# Autodesk Inventor assembly: Bird_wing_assembly
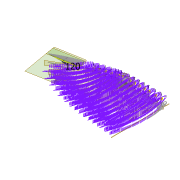
[picture p0: Inventor's stored thumbnail of the model, 180x180]
Saved by Autodesk Inventor 2022 (Build 260153000, 153)
## iProperties
Created: 2022-07-26
Part Number: Bird_wing_assembly
Document SubType Name: Assembly
Designer: dell
Mass: 478.578 g
Surface Area: 5047.89 cm^2
Volume: 478.578 cm^3
Density: 1 g/cm^3
Author: dell
## Documents named in this file (32)
- D:\xxxx\Uni\Part IV\MECHENG_700\Part_IV_project_CAD\Bird_skeleton_prototypes\Wing_drone_V1\Bird_wing_V2\Bird_wing_assembly.iam
- D:\xxxx\Uni\Part IV\MECHENG_700\Part_IV_project_CAD\Bird_skeleton_prototypes\Wing_drone_V1\Bird_wing_V2\Primary_hinge.ipt
- D:\xxxx\Uni\Part IV\MECHENG_700\Part_IV_project_CAD\Bird_skeleton_prototypes\Wing_drone_V1\Bird_wing_V2\Wing_arm_1.ipt
- D:\xxxx\Uni\Part IV\MECHENG_700\Part_IV_project_CAD\Bird_skeleton_prototypes\Wing_drone_V1\Bird_wing_V2\New_hinge_assembly.iam
- D:\xxxx\Uni\Part IV\MECHENG_700\Part_IV_project_CAD\Bird_skeleton_prototypes\Wing_drone_V1\Bird_wing_V2\Wing_arm_2.ipt
- D:\xxxx\Uni\Part IV\MECHENG_700\Part_IV_project_CAD\Bird_skeleton_prototypes\Wing_drone_V1\Bird_wing_V2\New_large_hinge_assembly.iam
- D:\xxxx\Uni\Part IV\MECHENG_700\Part_IV_project_CAD\Bird_skeleton_prototypes\Wing_drone_V1\Bird_wing_V2\Wing_arm_3.ipt
- D:\xxxx\Uni\Part IV\MECHENG_700\Part_IV_project_CAD\Bird_skeleton_prototypes\Wing_drone_V1\Bird_wing_V2\Arm_clip.ipt
- D:\xxxx\Uni\Part IV\MECHENG_700\Part_IV_project_CAD\Bird_skeleton_prototypes\Wing_drone_V1\Bird_wing_V2\Feather_clip.ipt
- D:\xxxx\Uni\Part IV\MECHENG_700\Part_IV_project_CAD\Bird_skeleton_prototypes\Wing_drone_V1\Bird_wing_V2\Feather_1\NACA_4412_300mm_feather_1_PLA.ipt
- D:\xxxx\Uni\Part IV\MECHENG_700\Part_IV_project_CAD\Bird_skeleton_prototypes\Wing_drone_V1\Bird_wing_V2\Feather_2\NACA_4412_300mm_feather_2_PLA.ipt
- D:\xxxx\Uni\Part IV\MECHENG_700\Part_IV_project_CAD\Bird_skeleton_prototypes\Wing_drone_V1\Bird_wing_V2\Feather_3\NACA_4412_340mm_feather_3_PLA.ipt
- D:\xxxx\Uni\Part IV\MECHENG_700\Part_IV_project_CAD\Bird_skeleton_prototypes\Wing_drone_V1\Bird_wing_V2\Feather_4\NACA_4412_340mm_feather_4_PLA.ipt
- D:\xxxx\Uni\Part IV\MECHENG_700\Part_IV_project_CAD\Bird_skeleton_prototypes\Wing_drone_V1\Bird_wing_V2\Feather_5\NACA_4412_340mm_feather_5_PLA.ipt
- D:\xxxx\Uni\Part IV\MECHENG_700\Part_IV_project_CAD\Bird_skeleton_prototypes\Wing_drone_V1\Bird_wing_V2\Feather_6\NACA_4412_340mm_feather_6_PLA.ipt
- D:\xxxx\Uni\Part IV\MECHENG_700\Part_IV_project_CAD\Bird_skeleton_prototypes\Wing_drone_V1\Bird_wing_V2\Feather_7\NACA_4412_340mm_feather_7_PLA.ipt
- D:\xxxx\Uni\Part IV\MECHENG_700\Part_IV_project_CAD\Bird_skeleton_prototypes\Wing_drone_V1\Bird_wing_V2\Feather_8\NACA_4412_340mm_feather_8_PLA.ipt
- D:\xxxx\Uni\Part IV\MECHENG_700\Part_IV_project_CAD\Bird_skeleton_prototypes\Wing_drone_V1\Bird_wing_V2\Feather_9\NACA_4412_340mm_feather_9_PLA.ipt
- D:\xxxx\Uni\Part IV\MECHENG_700\Part_IV_project_CAD\Bird_skeleton_prototypes\Wing_drone_V1\Bird_wing_V2\Feather_11\NACA_4412_340mm_feather_11_PLA.ipt
- D:\xxxx\Uni\Part IV\MECHENG_700\Part_IV_project_CAD\Bird_skeleton_prototypes\Wing_drone_V1\Bird_wing_V2\Feather_12\NACA_4412_340mm_feather_12_PLA.ipt
- D:\xxxx\Uni\Part IV\MECHENG_700\Part_IV_project_CAD\Bird_skeleton_prototypes\Wing_drone_V1\Bird_wing_V2\Feather_14\NACA_4412_340mm_feather_14_PLA.ipt
- D:\xxxx\Uni\Part IV\MECHENG_700\Part_IV_project_CAD\Bird_skeleton_prototypes\Wing_drone_V1\Bird_wing_V2\Feather_15\NACA_4412_340mm_feather_15_PLA.ipt
- D:\xxxx\Uni\Part IV\MECHENG_700\Part_IV_project_CAD\Bird_skeleton_prototypes\Wing_drone_V1\Bird_wing_V2\Feather_16\NACA_4412_340mm_feather_16_PLA.ipt
- D:\xxxx\Uni\Part IV\MECHENG_700\Part_IV_project_CAD\Bird_skeleton_prototypes\Wing_drone_V1\Bird_wing_V2\Feather_17\NACA_4412_340mm_feather_17_PLA.ipt
- D:\xxxx\Uni\Part IV\MECHENG_700\Part_IV_project_CAD\Bird_skeleton_prototypes\Wing_drone_V1\Bird_wing_V2\Wing_cover\Radius_joint_cover.ipt
- D:\xxxx\Uni\Part IV\MECHENG_700\Part_IV_project_CAD\Bird_skeleton_prototypes\Wing_drone_V1\Bird_wing_V2\Wing_cover\M4_nut.ipt
- D:\xxxx\Uni\Part IV\MECHENG_700\Part_IV_project_CAD\Bird_skeleton_prototypes\Wing_drone_V1\Bird_wing_V2\Wing_cover\Torsion_spring.ipt
- D:\xxxx\Uni\Part IV\MECHENG_700\Part_IV_project_CAD\Bird_skeleton_prototypes\Wing_drone_V1\Bird_wing_V2\Wing_cover\Manus_joint_cover.ipt
- D:\xxxx\Uni\Part IV\MECHENG_700\Part_IV_project_CAD\Bird_skeleton_prototypes\Wing_drone_V1\Bird_wing_V2\Wing_cover\Manus_joint_cover_2.ipt
- D:\xxxx\Uni\Part IV\MECHENG_700\Part_IV_project_CAD\Bird_skeleton_prototypes\Wing_drone_V1\Bird_wing_V2\Wing_cover\NACA_4412_500mm_cover.ipt
- D:\xxxx\Uni\Part IV\MECHENG_700\Part_IV_project_CAD\Bird_skeleton_prototypes\Wing_drone_V1\Bird_wing_V2\Primary_pulley_V2.ipt
- D:\xxxx\Uni\Part IV\MECHENG_700\Part_IV_project_CAD\Bird_skeleton_prototypes\Wing_drone_V1\Bird_wing_V2\Feather_0\Feather_0_assembly.iam
## Components (64 placed, 31 different names)
1. Primary_hinge:1 — Mate:1, Mate:2, Flush:1, Mate:3, Mate:4, Mate:5, Mate:158, Mate:160, Flush:31, Mate:179, Mate:180
2. Wing_arm_1:1 — Mate:3, Mate:4, Mate:5, Flush:10, Mate:67, Mate:68, Mate:108, Flush:27, Mate:109, Angle:19, Flush:29, Angle:20, Flush:30
3. Wing_arm_2:1 — Mate:14, Mate:16, Mate:15, Mate:69, Flush:11, Mate:70, Mate:87, Flush:13, Mate:89, Flush:15, Mate:90, Flush:16, Mate:106, Flush:21, Mate:107, Flush:22, Angle:12, Angle:14, Angle:15, Angle:17, Angle:18, Flush:33, Mate:168, Angle:26, Angle:28
4. New_hinge_assembly:3 [sub-assembly] — Mate:14, Mate:16, Mate:15, Mate:17, Mate:18, Angle:1, Flush:12, Flush:18, Flush:19, Flush:24, Flush:25, Angle:23
5. New_large_hinge_assembly:2 [sub-assembly] — Mate:17, Mate:18, Angle:1, Mate:19, Mate:20, Mate:21, Mate:39, Mate:40, Mate:46, Mate:51, Mate:52, Mate:58, Mate:62, Mate:66, Angle:21, Mate:164, Mate:165
6. Wing_arm_3:1 — Mate:19, Mate:20, Mate:21, Mate:25, Angle:2, Angle:3, Mate:38, Flush:3, Mate:43, Flush:4, Mate:47, Flush:5, Mate:50, Flush:6, Mate:55, Flush:7, Mate:61, Flush:8, Mate:65, Flush:9, Angle:5, Angle:6, Angle:7, Angle:8, Angle:9, Angle:10, Angle:11, Flush:32, Mate:181, Mate:182, Angle:27, Angle:28, Mate:185, Mate:186, Mate:187
7. Arm_clip:1 — Mate:25, Angle:2, Mate:27, Mate:28, Mate:39
8. Feather_clip:1 — Mate:27, Mate:28, Mate:35, Mate:36, Mate:37
9. NACA_4412_300mm_feather_1_PLA:1 — Mate:35, Mate:36, Mate:37, Angle:3
10. NACA_4412_340mm_feather_8_PLA:1 — Mate:125, Mate:126, Mate:127, Angle:11
11. Arm_clip:2 — Mate:38, Flush:3, Mate:40, Mate:41, Mate:42
12. Feather_clip:2 — Mate:41, Mate:42, Mate:73, Mate:74, Mate:75
13. Arm_clip:3 — Mate:43, Flush:4, Mate:44, Mate:45, Mate:46
14. Feather_clip:3 — Mate:44, Mate:45, Mate:110, Mate:111, Mate:112
15. Arm_clip:4 — Mate:47, Flush:5, Mate:48, Mate:49, Mate:51
16. Feather_clip:4 — Mate:48, Mate:49, Mate:113, Mate:114, Mate:115
17. Arm_clip:5 — Mate:50, Flush:6, Mate:52, Mate:53, Mate:54
18. Feather_clip:5 — Mate:53, Mate:54, Mate:116, Mate:117, Mate:118
19. Arm_clip:6 — Mate:55, Flush:7, Mate:56, Mate:57, Mate:58
20. Feather_clip:6 — Mate:56, Mate:57, Mate:119, Mate:120, Mate:121
21. Arm_clip:7 — Mate:61, Flush:8, Mate:62
22. Feather_clip:7 — Mate:122, Mate:123, Mate:124
23. Arm_clip:8 — Mate:65, Flush:9, Mate:66
24. Feather_clip:8 — Mate:125, Mate:126, Mate:127
25. New_hinge_assembly:4 [sub-assembly] — Flush:10, Mate:67, Mate:68, Mate:71, Mate:72, Angle:4, Mate:183, Mate:184
26. New_hinge_assembly:5 [sub-assembly] — Mate:69, Flush:11, Mate:70, Mate:71, Mate:72, Angle:4
27. NACA_4412_300mm_feather_2_PLA:1 — Mate:73, Mate:74, Mate:75, Angle:5
28. Arm_clip:9 — Mate:87, Flush:12, Flush:13
29. Feather_clip:9 — Mate:128, Mate:129, Mate:130
30. Arm_clip:11 — Mate:89, Flush:15, Flush:18
31. Feather_clip:11 — Mate:134, Mate:135, Mate:136
32. Arm_clip:12 — Mate:90, Flush:16, Flush:19
33. Feather_clip:12 — Mate:137, Mate:138, Mate:139
34. Arm_clip:14 — Mate:106, Flush:21, Flush:24
35. Feather_clip:14 — Mate:143, Mate:144, Mate:145
36. Arm_clip:15 — Mate:107, Flush:22, Flush:25
37. Feather_clip:15 — Mate:146, Mate:147, Mate:148
38. Arm_clip:16 — Mate:109, Flush:29, Mate:184
39. Feather_clip:16 — Mate:152, Mate:153, Mate:154
40. Arm_clip:17 — Mate:108, Flush:27, Mate:183
41. NACA_4412_340mm_feather_12_PLA:1 — Mate:137, Mate:138, Mate:139, Angle:15
42. Feather_clip:17 — Mate:149, Mate:150, Mate:151
43. NACA_4412_340mm_feather_3_PLA:1 — Mate:110, Mate:111, Mate:112, Angle:6
44. NACA_4412_340mm_feather_4_PLA:1 — Mate:113, Mate:114, Mate:115, Angle:7
45. NACA_4412_340mm_feather_5_PLA:1 — Mate:116, Mate:117, Mate:118, Angle:8
46. NACA_4412_340mm_feather_6_PLA:2 — Mate:119, Mate:120, Mate:121, Angle:9
47. NACA_4412_340mm_feather_7_PLA:1 — Mate:122, Mate:123, Mate:124, Angle:10
48. NACA_4412_340mm_feather_9_PLA:1 — Mate:128, Mate:129, Mate:130, Angle:12
49. NACA_4412_340mm_feather_11_PLA:1 — Mate:134, Mate:135, Mate:136, Angle:14
50. NACA_4412_340mm_feather_14_PLA:1 — Mate:143, Mate:144, Mate:145, Angle:17
51. NACA_4412_340mm_feather_15_PLA:1 — Mate:146, Mate:147, Mate:148, Angle:18
52. NACA_4412_340mm_feather_16_PLA:1 — Mate:149, Mate:150, Mate:151, Angle:19
53. NACA_4412_340mm_feather_17_PLA:1 — Mate:152, Mate:153, Mate:154, Angle:20
54. Radius_joint_cover:1 — Flush:30, Mate:160, Mate:161, Mate:178
55. M4_nut:1 — Mate:158
56. Torsion_spring:1 — Mate:161, Flush:31, Mate:178
57. Manus_joint_cover:1 — Angle:21, Flush:32, Mate:163, Mate:164
58. Manus_joint_cover_2:5 — Mate:165, Flush:33, Angle:23
59. NACA_4412_500mm_cover:1 — Mate:168, Angle:26
60. Primary_pulley_V2:1 — Mate:179, Mate:180
61. Feather_0_assembly:1 [sub-assembly] — Mate:181, Mate:182, Angle:27
62. NACA_4412_500mm_cover:2 — Mate:185
63. NACA_4412_500mm_cover:3 — Mate:187
64. NACA_4412_500mm_cover:4 — Mate:186
## Relationships (183: Mate 134, Flush 26, Angle 23)
- Mate:1: Primary_hinge:1
- Mate:2: Primary_hinge:1
- Flush:1: Primary_hinge:1
- Mate:3: Primary_hinge:1 ↔ Wing_arm_1:1
- Mate:4: Primary_hinge:1 ↔ Wing_arm_1:1
- Mate:5: Primary_hinge:1 ↔ Wing_arm_1:1
- Mate:14: Wing_arm_2:1 ↔ New_hinge_assembly:3
- Mate:16: Wing_arm_2:1 ↔ New_hinge_assembly:3
- Mate:15: Wing_arm_2:1 ↔ New_hinge_assembly:3
- Mate:17: New_hinge_assembly:3 ↔ New_large_hinge_assembly:2
- Mate:18 (0.1 mm): New_hinge_assembly:3 ↔ New_large_hinge_assembly:2
- Angle:1 (10 deg): New_hinge_assembly:3 ↔ New_large_hinge_assembly:2
- Mate:19: New_large_hinge_assembly:2 ↔ Wing_arm_3:1
- Mate:20: New_large_hinge_assembly:2 ↔ Wing_arm_3:1
- Mate:21: New_large_hinge_assembly:2 ↔ Wing_arm_3:1
- Mate:25: Wing_arm_3:1 ↔ Arm_clip:1
- Angle:2 (90 deg): Wing_arm_3:1 ↔ Arm_clip:1
- Mate:27: Arm_clip:1 ↔ Feather_clip:1
- Mate:28: Arm_clip:1 ↔ Feather_clip:1
- Mate:35: Feather_clip:1 ↔ NACA_4412_300mm_feather_1_PLA:1
- Mate:36: Feather_clip:1 ↔ NACA_4412_300mm_feather_1_PLA:1
- Mate:37 (0.1 mm): Feather_clip:1 ↔ NACA_4412_300mm_feather_1_PLA:1
- Angle:3 (160 deg): Wing_arm_3:1 ↔ NACA_4412_300mm_feather_1_PLA:1
- Mate:38: Wing_arm_3:1 ↔ Arm_clip:2
- Flush:3: Wing_arm_3:1 ↔ Arm_clip:2
- Mate:39 (310 mm): New_large_hinge_assembly:2 ↔ Arm_clip:1
- Mate:40 (260 mm): New_large_hinge_assembly:2 ↔ Arm_clip:2
- Mate:41: Arm_clip:2 ↔ Feather_clip:2
- Mate:42: Arm_clip:2 ↔ Feather_clip:2
- Mate:43: Wing_arm_3:1 ↔ Arm_clip:3
- Flush:4: Wing_arm_3:1 ↔ Arm_clip:3
- Mate:44: Arm_clip:3 ↔ Feather_clip:3
- Mate:45: Arm_clip:3 ↔ Feather_clip:3
- Mate:46 (210 mm): New_large_hinge_assembly:2 ↔ Arm_clip:3
- Mate:47: Wing_arm_3:1 ↔ Arm_clip:4
- Flush:5: Wing_arm_3:1 ↔ Arm_clip:4
- Mate:48: Arm_clip:4 ↔ Feather_clip:4
- Mate:49: Arm_clip:4 ↔ Feather_clip:4
- Mate:50: Wing_arm_3:1 ↔ Arm_clip:5
- Flush:6: Wing_arm_3:1 ↔ Arm_clip:5
- Mate:51 (160 mm): New_large_hinge_assembly:2 ↔ Arm_clip:4
- Mate:52 (110 mm): New_large_hinge_assembly:2 ↔ Arm_clip:5
- Mate:53: Arm_clip:5 ↔ Feather_clip:5
- Mate:54: Arm_clip:5 ↔ Feather_clip:5
- Mate:55: Wing_arm_3:1 ↔ Arm_clip:6
- Flush:7: Wing_arm_3:1 ↔ Arm_clip:6
- Mate:56: Arm_clip:6 ↔ Feather_clip:6
- Mate:57: Arm_clip:6 ↔ Feather_clip:6
- Mate:58 (70 mm): New_large_hinge_assembly:2 ↔ Arm_clip:6
- [Mate]: Arm_clip:7 ↔ Feather_clip:7
- [Mate]: Arm_clip:7 ↔ Feather_clip:7
- Mate:61: Wing_arm_3:1 ↔ Arm_clip:7
- Flush:8: Wing_arm_3:1 ↔ Arm_clip:7
- Mate:62 (40 mm): New_large_hinge_assembly:2 ↔ Arm_clip:7
- [Mate]: Arm_clip:8 ↔ Feather_clip:8
- [Mate]: Arm_clip:8 ↔ Feather_clip:8
- Mate:65: Wing_arm_3:1 ↔ Arm_clip:8
- Flush:9: Wing_arm_3:1 ↔ Arm_clip:8
- Mate:66 (10 mm): New_large_hinge_assembly:2 ↔ Arm_clip:8
- Flush:10: Wing_arm_1:1 ↔ New_hinge_assembly:4
- Mate:67: Wing_arm_1:1 ↔ New_hinge_assembly:4
- Mate:68: Wing_arm_1:1 ↔ New_hinge_assembly:4
- Mate:69: Wing_arm_2:1 ↔ New_hinge_assembly:5
- Flush:11: Wing_arm_2:1 ↔ New_hinge_assembly:5
- Mate:70: Wing_arm_2:1 ↔ New_hinge_assembly:5
- Mate:71: New_hinge_assembly:4 ↔ New_hinge_assembly:5
- Mate:72 (0.1 mm): New_hinge_assembly:4 ↔ New_hinge_assembly:5
- Angle:4 (0 deg): New_hinge_assembly:4 ↔ New_hinge_assembly:5
- Mate:73: Feather_clip:2 ↔ NACA_4412_300mm_feather_2_PLA:1
- Mate:74: Feather_clip:2 ↔ NACA_4412_300mm_feather_2_PLA:1
- Mate:75 (0.1 mm): Feather_clip:2 ↔ NACA_4412_300mm_feather_2_PLA:1
- Angle:5 (140 deg): Wing_arm_3:1 ↔ NACA_4412_300mm_feather_2_PLA:1
- [Mate]: Arm_clip:9 ↔ Feather_clip:9
- [Mate]: Arm_clip:9 ↔ Feather_clip:9
- [Mate]: Arm_clip:11 ↔ Feather_clip:11
- [Mate]: Arm_clip:11 ↔ Feather_clip:11
- [Mate]: Arm_clip:12 ↔ Feather_clip:12
- [Mate]: Arm_clip:12 ↔ Feather_clip:12
- Mate:87: Wing_arm_2:1 ↔ Arm_clip:9
- Flush:12 (-10 mm): New_hinge_assembly:3 ↔ Arm_clip:9
- Flush:13: Wing_arm_2:1 ↔ Arm_clip:9
- Mate:89: Wing_arm_2:1 ↔ Arm_clip:11
- Flush:15: Wing_arm_2:1 ↔ Arm_clip:11
- Mate:90: Wing_arm_2:1 ↔ Arm_clip:12
- Flush:16: Wing_arm_2:1 ↔ Arm_clip:12
- Flush:18 (-58 mm): New_hinge_assembly:3 ↔ Arm_clip:11
- Flush:19 (-106 mm): New_hinge_assembly:3 ↔ Arm_clip:12
- [Mate]: Arm_clip:14 ↔ Feather_clip:14
- [Mate]: Arm_clip:14 ↔ Feather_clip:14
- [Mate]: Arm_clip:15 ↔ Feather_clip:15
- [Mate]: Arm_clip:15 ↔ Feather_clip:15
- [Mate]: Arm_clip:16 ↔ Feather_clip:16
- [Mate]: Arm_clip:16 ↔ Feather_clip:16
- [Mate]: Arm_clip:17 ↔ Feather_clip:17
- [Mate]: Arm_clip:17 ↔ Feather_clip:17
- Mate:106: Wing_arm_2:1 ↔ Arm_clip:14
- Flush:21: Wing_arm_2:1 ↔ Arm_clip:14
- Mate:107: Wing_arm_2:1 ↔ Arm_clip:15
- Flush:22: Wing_arm_2:1 ↔ Arm_clip:15
- Flush:24 (-154 mm): New_hinge_assembly:3 ↔ Arm_clip:14
- Flush:25 (-202 mm): New_hinge_assembly:3 ↔ Arm_clip:15
- Mate:108: Wing_arm_1:1 ↔ Arm_clip:17
- Flush:27: Wing_arm_1:1 ↔ Arm_clip:17
- Mate:109: Wing_arm_1:1 ↔ Arm_clip:16
- Mate:110: Feather_clip:3 ↔ NACA_4412_340mm_feather_3_PLA:1
- Mate:111: Feather_clip:3 ↔ NACA_4412_340mm_feather_3_PLA:1
- Mate:112 (0.1 mm): Feather_clip:3 ↔ NACA_4412_340mm_feather_3_PLA:1
- Angle:6 (130 deg): Wing_arm_3:1 ↔ NACA_4412_340mm_feather_3_PLA:1
- Mate:113: Feather_clip:4 ↔ NACA_4412_340mm_feather_4_PLA:1
- Mate:114: Feather_clip:4 ↔ NACA_4412_340mm_feather_4_PLA:1
- Mate:115 (0.1 mm): Feather_clip:4 ↔ NACA_4412_340mm_feather_4_PLA:1
- Angle:7 (238 deg): Wing_arm_3:1 ↔ NACA_4412_340mm_feather_4_PLA:1
- Mate:116: Feather_clip:5 ↔ NACA_4412_340mm_feather_5_PLA:1
- Mate:117: Feather_clip:5 ↔ NACA_4412_340mm_feather_5_PLA:1
- Mate:118 (0.1 mm): Feather_clip:5 ↔ NACA_4412_340mm_feather_5_PLA:1
- Mate:119: Feather_clip:6 ↔ NACA_4412_340mm_feather_6_PLA:2
- Mate:120: Feather_clip:6 ↔ NACA_4412_340mm_feather_6_PLA:2
- Mate:121 (0.1 mm): Feather_clip:6 ↔ NACA_4412_340mm_feather_6_PLA:2
- Mate:122: Feather_clip:7 ↔ NACA_4412_340mm_feather_7_PLA:1
- Mate:123: Feather_clip:7 ↔ NACA_4412_340mm_feather_7_PLA:1
- Mate:124 (0.1 mm): Feather_clip:7 ↔ NACA_4412_340mm_feather_7_PLA:1
- Angle:8 (242 deg): Wing_arm_3:1 ↔ NACA_4412_340mm_feather_5_PLA:1
- Angle:9 (247 deg): Wing_arm_3:1 ↔ NACA_4412_340mm_feather_6_PLA:2
- Angle:10 (255 deg): Wing_arm_3:1 ↔ NACA_4412_340mm_feather_7_PLA:1
- Mate:125: NACA_4412_340mm_feather_8_PLA:1 ↔ Feather_clip:8
- Mate:126: NACA_4412_340mm_feather_8_PLA:1 ↔ Feather_clip:8
- Mate:127 (0.1 mm): NACA_4412_340mm_feather_8_PLA:1 ↔ Feather_clip:8
- Angle:11 (100 deg): Wing_arm_3:1 ↔ NACA_4412_340mm_feather_8_PLA:1
- Mate:128: Feather_clip:9 ↔ NACA_4412_340mm_feather_9_PLA:1
- Mate:129: Feather_clip:9 ↔ NACA_4412_340mm_feather_9_PLA:1
- Mate:130 (0.1 mm): Feather_clip:9 ↔ NACA_4412_340mm_feather_9_PLA:1
- Angle:12 (95 deg): Wing_arm_2:1 ↔ NACA_4412_340mm_feather_9_PLA:1
- Mate:134: Feather_clip:11 ↔ NACA_4412_340mm_feather_11_PLA:1
- Mate:135: Feather_clip:11 ↔ NACA_4412_340mm_feather_11_PLA:1
- Mate:136 (0.1 mm): Feather_clip:11 ↔ NACA_4412_340mm_feather_11_PLA:1
- Angle:14 (268 deg): Wing_arm_2:1 ↔ NACA_4412_340mm_feather_11_PLA:1
- Mate:137: Feather_clip:12 ↔ NACA_4412_340mm_feather_12_PLA:1
- Mate:138: Feather_clip:12 ↔ NACA_4412_340mm_feather_12_PLA:1
- Mate:139 (0.1 mm): Feather_clip:12 ↔ NACA_4412_340mm_feather_12_PLA:1
- Angle:15 (269 deg): Wing_arm_2:1 ↔ NACA_4412_340mm_feather_12_PLA:1
- Mate:143: Feather_clip:14 ↔ NACA_4412_340mm_feather_14_PLA:1
- Mate:144: Feather_clip:14 ↔ NACA_4412_340mm_feather_14_PLA:1
- Mate:145 (0.1 mm): Feather_clip:14 ↔ NACA_4412_340mm_feather_14_PLA:1
- Angle:17 (269 deg): Wing_arm_2:1 ↔ NACA_4412_340mm_feather_14_PLA:1
- Mate:146: Feather_clip:15 ↔ NACA_4412_340mm_feather_15_PLA:1
- Mate:147: Feather_clip:15 ↔ NACA_4412_340mm_feather_15_PLA:1
- Mate:148 (0.1 mm): Feather_clip:15 ↔ NACA_4412_340mm_feather_15_PLA:1
- Angle:18 (90 deg): Wing_arm_2:1 ↔ NACA_4412_340mm_feather_15_PLA:1
- Mate:149: Feather_clip:17 ↔ NACA_4412_340mm_feather_16_PLA:1
- Mate:150: Feather_clip:17 ↔ NACA_4412_340mm_feather_16_PLA:1
- Mate:151 (0.1 mm): Feather_clip:17 ↔ NACA_4412_340mm_feather_16_PLA:1
- Angle:19 (270 deg): Wing_arm_1:1 ↔ NACA_4412_340mm_feather_16_PLA:1
- Mate:152: Feather_clip:16 ↔ NACA_4412_340mm_feather_17_PLA:1
- Mate:153: Feather_clip:16 ↔ NACA_4412_340mm_feather_17_PLA:1
- Mate:154 (0.1 mm): Feather_clip:16 ↔ NACA_4412_340mm_feather_17_PLA:1
- Flush:29: Wing_arm_1:1 ↔ Arm_clip:16
- Angle:20 (90 deg): Wing_arm_1:1 ↔ NACA_4412_340mm_feather_17_PLA:1
- Mate:158: Primary_hinge:1 ↔ M4_nut:1
- Flush:30: Wing_arm_1:1 ↔ Radius_joint_cover:1
- Mate:160: Primary_hinge:1 ↔ Radius_joint_cover:1
- Mate:161: Radius_joint_cover:1 ↔ Torsion_spring:1
- Flush:31: Primary_hinge:1 ↔ Torsion_spring:1
- Angle:21 (10 deg): New_large_hinge_assembly:2 ↔ Manus_joint_cover:1
- Flush:32: Wing_arm_3:1 ↔ Manus_joint_cover:1
- Mate:163: Manus_joint_cover:1
- Mate:164: New_large_hinge_assembly:2 ↔ Manus_joint_cover:1
- Mate:165: New_large_hinge_assembly:2 ↔ Manus_joint_cover_2:5
- Flush:33: Wing_arm_2:1 ↔ Manus_joint_cover_2:5
- Angle:23 (-60 deg): New_hinge_assembly:3 ↔ Manus_joint_cover_2:5
- Mate:168: Wing_arm_2:1 ↔ NACA_4412_500mm_cover:1
- Angle:26 (0 deg): Wing_arm_2:1 ↔ NACA_4412_500mm_cover:1
- Mate:178: Radius_joint_cover:1 ↔ Torsion_spring:1
- Mate:179: Primary_hinge:1 ↔ Primary_pulley_V2:1
- Mate:180: Primary_hinge:1 ↔ Primary_pulley_V2:1
- Mate:181: Wing_arm_3:1 ↔ Feather_0_assembly:1
- Mate:182: Wing_arm_3:1 ↔ Feather_0_assembly:1
- Angle:27 (0 deg): Wing_arm_3:1 ↔ Feather_0_assembly:1
- Mate:183 (12 mm): New_hinge_assembly:4 ↔ Arm_clip:17
- Mate:184 (72 mm): New_hinge_assembly:4 ↔ Arm_clip:16
- Angle:28 (-10 deg): Wing_arm_2:1 ↔ Wing_arm_3:1
- Mate:185: Wing_arm_3:1 ↔ NACA_4412_500mm_cover:2
- Mate:186: Wing_arm_3:1 ↔ NACA_4412_500mm_cover:4
- Mate:187: Wing_arm_3:1 ↔ NACA_4412_500mm_cover:3
## Named parameters: d109_d106 = 0 mm, d110_d107 = 0 mm, d114_d109_d106 = 0 mm, d115_d110_d107 = 0 mm, d138_d114_d109_d106 = 0 mm, d139_d115_d110_d107 = 0 mm, d142_d114_d109_d106 = 0 mm, d143_d115_d110_d107 = 0 mm, d144_d114_d109_d106 = 0 mm, d145_d115_d110_d107 = 0 mm, d160_d144_d114_d109_d106 = 0 mm, d161_d145_d115_d110_d107 = 0 mm, d162_d144_d114_d109_d106 = 0 mm, d163_d145_d115_d110_d107 = 0 mm, d164_d144_d114_d109_d106 = 0 mm, d165_d145_d115_d110_d107 = 0 mm, d166_d144_d114_d109_d106 = 0 mm, d167_d145_d115_d110_d107 = 0 mm
